# Autodesk Inventor assembly: Turret Base
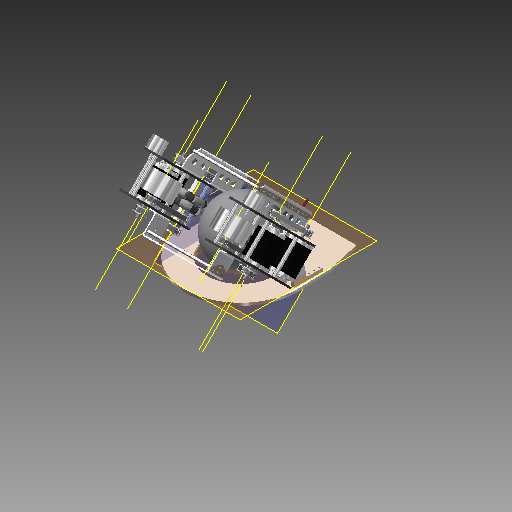
[picture p0: Inventor's stored thumbnail of the model, 512x512]
Saved by Autodesk Inventor 2019.4 (Build 234330000, 330)
## iProperties
Created: 2020-01-06
Part Number: Turret Base
Document SubType Name: Assembly
Designer: admin
Mass: 10071.2 g
Surface Area: 14374.3 cm^2
Volume: 7031.95 cm^3
Density: 1.43221 g/cm^3
Author: admin
## Documents named in this file (9)
- C:\Users\Mark\Desktop\7738 Helion Engineering\7738-2020\Turret\Turret Base.iam
- C:\Users\Mark\Desktop\7738 Helion Engineering\7738-2020\Turret\Slewing Bearing.ipt
- C:\Users\Mark\Desktop\7738 Helion Engineering\7738-2020\Turret\Turret Base Plate.ipt
- C:\Users\Mark\Desktop\7738 Helion Engineering\7738-2020\CAD\Gearbox\F6804.ipt
- C:\Users\Mark\Desktop\7738 Helion Engineering\7738-2020\Turret\Turret Shooter Assembly.iam
- C:\Users\Mark\Desktop\7738 Helion Engineering\7738-2020\Turret\Idle Shooter holder.ipt
- C:\Users\Mark\Desktop\7738 Helion Engineering\7738-2020\Turret\Bearing Shooter Holder.ipt
- C:\Users\Mark\Desktop\7738 Helion Engineering\7738-2020\Turret\Turret Base\Design Accelerator\Chain Drive2.iam
- C:\Users\Mark\Desktop\7738 Helion Engineering\7738-2020\Turret\Gearbox+Motor\VersaPlanetary_v2_Two_Stage_100_1_with_BAG.iam
## Components (9 placed, 8 different names)
1. Slewing Bearing:1 — Mate:1, Mate:2, Mate:5, Mate:6, Mate:25, Mate:36, Mate:37, Mate:38
2. Turret Base Plate:1 — Mate:5, Mate:6, Angle:2, Mate:26, Angle:3, Mate:29, Mate:34, Flush:1, Mate:39
3. F6804:2 — Mate:31, Mate:32, Mate:33
4. Turret Shooter Assembly:1 [sub-assembly] — Mate:25, Angle:3, Angle:4, Mate:27, Mate:28, Mate:30, Mate:33
5. Idle Shooter holder:1 — Mate:26, Mate:27, Mate:28
6. Bearing Shooter Holder:1 — Mate:29, Mate:30, Mate:31, Mate:32
7. Chain Drive:1 [sub-assembly] — Mate:35
8. VersaPlanetary_v2_Two_Stage_100_1_with_BAG:1 [sub-assembly] — Mate:34, Mate:35
9. Slewing Bearing:2 — Mate:36, Mate:37, Mate:38, Mate:39
## Relationships (23: Mate 19, Angle 3, Flush 1)
- Mate:1: Slewing Bearing:1
- Mate:2: Slewing Bearing:1
- Mate:5: Slewing Bearing:1 ↔ Turret Base Plate:1
- Mate:6: Slewing Bearing:1 ↔ Turret Base Plate:1
- Angle:2 (180 deg): Turret Base Plate:1
- Mate:25: Slewing Bearing:1 ↔ Turret Shooter Assembly:1
- Mate:26: Turret Base Plate:1 ↔ Idle Shooter holder:1
- Angle:3 (225 deg): Turret Base Plate:1 ↔ Turret Shooter Assembly:1
- Angle:4 (180 deg): Turret Shooter Assembly:1
- Mate:27: Turret Shooter Assembly:1 ↔ Idle Shooter holder:1
- Mate:28 (1.1 mm): Turret Shooter Assembly:1 ↔ Idle Shooter holder:1
- Mate:29: Turret Base Plate:1 ↔ Bearing Shooter Holder:1
- Mate:30: Turret Shooter Assembly:1 ↔ Bearing Shooter Holder:1
- Mate:31: F6804:2 ↔ Bearing Shooter Holder:1
- Mate:32 (0.2 mm): F6804:2 ↔ Bearing Shooter Holder:1
- Mate:33 (1.1 mm): F6804:2 ↔ Turret Shooter Assembly:1
- Mate:34: Turret Base Plate:1 ↔ VersaPlanetary_v2_Two_Stage_100_1_with_BAG:1
- Flush:1 (22.225 mm): Turret Base Plate:1
- Mate:35: Chain Drive:1 ↔ VersaPlanetary_v2_Two_Stage_100_1_with_BAG:1
- Mate:36: Slewing Bearing:1 ↔ Slewing Bearing:2
- Mate:37: Slewing Bearing:1 ↔ Slewing Bearing:2
- Mate:38: Slewing Bearing:1 ↔ Slewing Bearing:2
- Mate:39: Turret Base Plate:1 ↔ Slewing Bearing:2
